# Autodesk Inventor assembly: CJ2B10-100Z(0_1_0)
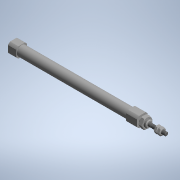
[picture p0: Inventor's stored thumbnail of the model, 180x180]
Saved by Autodesk Inventor 2022.3 (Build 263350000, 350)
## iProperties
Category: PARTsolutions
Company: SMC
Part Number: CJ2B10-100Z(0_1_0)
Catalog Web Link: www.cadenas.de
Description: CJ2-Z/CDJ2-Z-Air Cylinder/Standard: Double Acting Single Rod
Vendor: SMC
Document SubType Name: Assembly
Designer: partserver
Manufacturer: SMC
Mass: 9.11356 g
Surface Area: 122.894 cm^2
Volume: 9.11356 cm^3
Density: 1 g/cm^3
PSOL_IDENT_0: {$CADENAS_DATA\23d-libs\smc_jp\actuator\standard_air_cylinder\cj2\cj2_z_asmtab.prj},309 {VTYP=3D},{S
PSOL_IDENT_1: TYP=ASSTAB},{NB=CJ2B10-100Z(0_1_0)},{LINA=CJ2B10-100Z},{NN=CJ2-Z/CDJ2-Z},{DATE=02.02.2022 09:27:27},
PSOL_IDENT_2: {GEOMDATE=16.09.2020 08:28:58},{VERSION=},{LINEID=370},{WBVAR=MAGNET,AUTOSWITCH,LEAD,NUMBER,CUSHION,
PSOL_IDENT_3: STROKE,POS,PORT,STOP,BRACKET,RODB,MOUNTING,OMSC,OMSCXC3,OMSCXC51,THREAD},{WBNUMERIC=STROKE,POS}  {NB=
PSOL_IDENT_4: CJ2B10-100Z(0_1_0)},{LINA=CJ2B10-100Z},{KT=DUMMY},{NENN=CJ2B10-100Z},{ORDER=CJ2B10-100Z},{BORE=10},{
PSOL_IDENT_5: MOUNT=(B) Basic},{MOUNTX=B},{MAGNET=},{AUTOSWITCH=},{AUTOSWX='','N/A'},{LEAD=},{LEADX= '','N/A' },{N
PSOL_IDENT_6: UMBER=},{CUSHION=},{CUSHIONX= '','(-) Rubber cushion','A','(A) Air cushion' },{SWSIGNX= '','N/A' },{
PSOL_IDENT_7: STROKE=100},{STDSTROKE=<75>,15,30,45,60,75,100,125,150},{STROKE1X=[2:400/1]},{SMIN=2},{SMINASW1=10},
PSOL_IDENT_8: {SMINASW2=15},{SMAX1=400},{POS=0},{PORT=},{STOP=1},{COM=Please confirm the conditions of use with SM
PSOL_IDENT_9: C},{COM1=-},{BRACKET=},{RODB=},{RODBX= '', '(-) None', 'V', '(V) Single knuckle joint', 'W'  , '(W)
PSOL_IDENT_10: Double knuckle joint', 'T', '(T) Rod end cap (Flat type)', 'U'  , '(U) Rod end cap (Round type)' },{
PSOL_IDENT_11: MOUNTING=},{OMSC=},{OMSCXC3=},{OMSCXC51=},{THREAD=0},{MOUNTINGX='','N/A'},{BRACKETX='','N/A'},{PORTX=''
PSOL_IDENT_12: , '(-) Perpendicular to axis', 'R', '(R) Axial'},{SW=B},{OMSCX= '','(-) None','-XB6','(XB6) Heat res
PSOL_IDENT_13: istant cylinder (-10 to 150 degree Celsius)','-XB7','(XB7) Cold resistant cylinder (-40 to 70 degree
PSOL_IDENT_14: Celsius)','-XB9','(XB9) Low speed cylinder (10 to 50 mm/s)','-XC22','(XC22) Fluororubber seals','-X
PSOL_IDENT_15: C85','(XC85) Grease specification for food processing machines', '-X446'  , '(X446) PTFE grease' },{
PSOL_IDENT_16: A=2.5},{XC3= '','(-) None','-XC3AB','(XC3AB) Rod port location viewed: A,Head port location viewed:
PSOL_IDENT_17: B','-XC3AC','(XC3AC) Rod port location viewed: A,Head port location viewed: C','-XC3AD','(XC3AD) Rod
PSOL_IDENT_18: port location viewed: A,Head port location viewed: D','-XC3BA','(XC3BA) Rod port location viewed: B
PSOL_IDENT_19: ,Head port location viewed: A','-XC3BB','(XC3BB) Rod port location viewed: B,Head port location view
PSOL_IDENT_20: ed: B','-XC3BC','(XC3BC) Rod port location viewed: B,Head port location viewed: C','-XC3BD','(XC3BD)
PSOL_IDENT_21: Rod port location viewed: B,Head port location viewed: D','-XC3CA','(XC3CA) Rod port location viewe
PSOL_IDENT_22: d: C,Head port location viewed: A','-XC3CB','(XC3CB) Rod port location viewed: C,Head port location
PSOL_IDENT_23: viewed: B','-XC3CC','(XC3CC) Rod port location viewed: C,Head port location viewed: C','-XC3CD','(XC
PSOL_IDENT_24: 3CD) Rod port location viewed: C,Head port location viewed: D','-XC3DA','(XC3DA) Rod port location v
PSOL_IDENT_25: iewed: D,Head port location viewed: A','-XC3DB','(XC3DB) Rod port location viewed: D,Head port locat
PSOL_IDENT_26: ion viewed: B','-XC3DC','(XC3DC) Rod port location viewed: D,Head port location viewed: C','-XC3DD','
PSOL_IDENT_27: (XC3DD) Rod port location viewed: D,Head port location viewed: D' },{XC51= '','(-) None','-XC51H4','
PSOL_IDENT_28: (XC51H4) Hose nipple type: ø4/2.5 with restriction','-XC51H6','(XC51H6) Hose nipple type: ø6/4 with
PSOL_IDENT_29: restriction','-XC51MH4','(XC51MH4) Hose nipple type: ø4/2.5 without restriction','-XC51MH6','(XC51MH
PSOL_IDENT_30: 6) Hose nipple type: ø6/4 without restriction' },{BMP=B},{PPATH=cj2_z/assembly/cj2_z_asmsbl.prj},{OM
PSOL_IDENT_31: SCXX= '','(-) None','-XB6','(XB6) Heat resistant cylinder (-10 to 150 degree Celsius)','-XB7','(XB7)
PSOL_IDENT_32: Cold resistant cylinder (-40 to 70 degree Celsius)','-XB9','(XB9) Low speed cylinder (10 to 50 mm/s
PSOL_IDENT_33: )','-XC22','(XC22) Fluororubber seals','-XC85','(XC85) Grease specification for food processing mach
PSOL_IDENT_34: ines', '-X446'  , '(X446) PTFE grease' }
NB: CJ2B10-100Z(0_1_0)
NN: CJ2-Z/CDJ2-Z
NT: Air Cylinder/Standard: Double Acting Single Rod
NBSYN: $ORDER.($POS._$STOP._$THREAD.)
LINA: CJ2B10-100Z
CATALOG: SMC (JP
BORE: 10
MOUNT: (B) Basic
MAGNET: (-) Without magnet
AUTOSWITCH: N/A
LEAD: N/A
NUMBER: N/A
CUSHION: (-) Rubber cushion
STROKE: 100
POS: 0
PORT: (-) Perpendicular to axis
STOP: Manufacturable stroke
COM: Please confirm the conditions of use with SMC
COM1: -
BRACKET: N/A
RODB: (-) None
MOUNTING: N/A
OMSC: (-) None
OMSCXC3: (-) None
OMSCXC51: (-) None
THREAD: on
SUPPLIER: SMC
ARTICLENO: CJ2B10-100Z(0_1_0)
BOMINFO: CJ2B10-100Z
CREATOR: CADENAS GmbH
Title: CJ2B10-100Z
Author: Cadenas PARTsolutions
Comments: Air Cylinder/Standard: Double Acting Single Rod
## Documents named in this file (5)
- C:\Users\YusukeKunita\Documents\GrabCAD\Development\BasicParts\AirCylinder\CJ2B10-100Z\CJ2B10-100Z.iam
- C:\Users\YusukeKunita\Documents\GrabCAD\Development\BasicParts\AirCylinder\CJ2B10-100Z\CJ2B10-100Z_BODY.ipt
- C:\Users\YusukeKunita\Documents\GrabCAD\Development\BasicParts\AirCylinder\CJ2B10-100Z\CJ2B10-100Z_ROD.ipt
- C:\Users\YusukeKunita\Documents\GrabCAD\Development\BasicParts\AirCylinder\CJ2B10-100Z\NTJ-010C.ipt
- C:\Users\YusukeKunita\Documents\GrabCAD\Development\BasicParts\AirCylinder\CJ2B10-100Z\SNJ-010C.ipt
## Components (5 placed, 4 different names)
1. CJ2B10-100Z_BODY:1 — body_Z@1 <-> ROD_BODY_Z@2, body_YZ@1 <-> ROD_BODY_YZ@2, body_XY@1 <-> ntj_XY@5, body_Z@1 <-> ntj_Z@5, body_YZ@1 <-> ntj_YZ@5, フラッシュ:3
2. CJ2B10-100Z_ROD:1 — body_Z@1 <-> ROD_BODY_Z@2, body_YZ@1 <-> ROD_BODY_YZ@2, rodnt1_XY@2 <-> ntj_XY@3, rodnt1_Z@2 <-> ntj_Z@3, rodnt1_YZ@2 <-> ntj_YZ@3, rodnt1_XY@2 <-> ntj_XY@4, rodnt1_Z@2 <-> ntj_Z@4, rodnt1_YZ@2 <-> ntj_YZ@4, フラッシュ:3
3. NTJ-010C:1 — rodnt1_XY@2 <-> ntj_XY@3, rodnt1_Z@2 <-> ntj_Z@3, rodnt1_YZ@2 <-> ntj_YZ@3
4. NTJ-010C:2 — rodnt1_XY@2 <-> ntj_XY@4, rodnt1_Z@2 <-> ntj_Z@4, rodnt1_YZ@2 <-> ntj_YZ@4
5. SNJ-010C:1 — body_XY@1 <-> ntj_XY@5, body_Z@1 <-> ntj_Z@5, body_YZ@1 <-> ntj_YZ@5
## Relationships (12: Mate 5, Angle 4, Flush 3)
- body_Z@1 <-> ROD_BODY_Z@2 [Mate]: CJ2B10-100Z_BODY:1 ↔ CJ2B10-100Z_ROD:1
- body_YZ@1 <-> ROD_BODY_YZ@2 [Angle] (0 deg): CJ2B10-100Z_BODY:1 ↔ CJ2B10-100Z_ROD:1
- rodnt1_XY@2 <-> ntj_XY@3 [Mate] (0.5 mm): CJ2B10-100Z_ROD:1 ↔ NTJ-010C:1
- rodnt1_Z@2 <-> ntj_Z@3 [Mate]: CJ2B10-100Z_ROD:1 ↔ NTJ-010C:1
- rodnt1_YZ@2 <-> ntj_YZ@3 [Angle] (0 deg): CJ2B10-100Z_ROD:1 ↔ NTJ-010C:1
- rodnt1_XY@2 <-> ntj_XY@4 [Flush]: CJ2B10-100Z_ROD:1 ↔ NTJ-010C:2
- rodnt1_Z@2 <-> ntj_Z@4 [Mate]: CJ2B10-100Z_ROD:1 ↔ NTJ-010C:2
- rodnt1_YZ@2 <-> ntj_YZ@4 [Angle] (0 deg): CJ2B10-100Z_ROD:1 ↔ NTJ-010C:2
- body_XY@1 <-> ntj_XY@5 [Flush] (-1.6 mm): CJ2B10-100Z_BODY:1 ↔ SNJ-010C:1
- body_Z@1 <-> ntj_Z@5 [Mate]: CJ2B10-100Z_BODY:1 ↔ SNJ-010C:1
- body_YZ@1 <-> ntj_YZ@5 [Angle] (0 deg): CJ2B10-100Z_BODY:1 ↔ SNJ-010C:1
- フラッシュ:3 [Flush] (-119.5 mm): CJ2B10-100Z_BODY:1 ↔ CJ2B10-100Z_ROD:1
